# Autodesk Inventor assembly: 2016-02-05-RhinoRobotV10
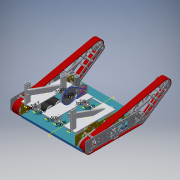
[picture p0: Inventor's stored thumbnail of the model, 180x180]
Saved by Autodesk Inventor 2016 SP1 (Build 200210100, 210)
## iProperties
Created: 2016-01-23
Part Number: 2016-02-05-RhinoRobotV10
Document SubType Name: Assembly
Designer: steele
Mass: 23360.3 g
Surface Area: 43274.3 cm^2
Volume: 23034.6 cm^3
Density: 1.01414 g/cm^3
Author: steele
## Documents named in this file (9)
- C:\snobotics\CAD-Development\robSteele\SnoBotics2016\2015-02-05-RhinoRobotNarrowView\2016-02-05-RhinoRobotV10.iam
- C:\snobotics\CAD-Development\robSteele\SnoBotics2016\RhinoTrackDriveModule\am-3322+RhinoTrackDriveModule.iam
- C:\snobotics\CAD-Development\robSteele\SnoBotics2016\RhinoBottomFloorOptions\RhinoBottomFloorPlate01.ipt
- C:\snobotics\CAD-Development\robSteele\SnoBotics2016\RhinoTrackDriveModule\am-3322+RhinoTrackDriveModule_MIR9.iam
- C:\snobotics\CAD-Development\robSteele\SnoBotics2016\AM Parts\Churo_16_5_inches.ipt
- C:\snobotics\CAD-Development\robSteele\SnoBotics2016\2016-01-31-Lift\ShortSupportPlateAssembly.iam
- C:\snobotics\CAD-Development\robSteele\SnoBotics2016\2015-02-05-RhinoRobotNarrowView\2016-02-05-RhinoRobotV10\Design Accelerator\Bolted Connection1.iam
- C:\snobotics\CAD-Development\robSteele\SnoBotics2016\2016-01-31-Lift\LongSupportPlateAssembly.iam
- C:\snobotics\CAD-Development\robSteele\SnoBotics2016\2016-01-31-Lift\ShortSupportPlateAssembly_MIR.iam
## Components (10 placed, 8 different names)
1. RhinoBottomFloorPlate01:1 — Mate:1, Flush:2, Flush:11
2. am-3322+RhinoTrackDriveModule:1 [sub-assembly] — Mate:1, Flush:2, Flush:11, Insert:1, Insert:2, Insert:6
3. am-3322+RhinoTrackDriveModule_MIR9:1 [sub-assembly]
4. Churo_16_5_inches:1 — Insert:1, Flush:18, Insert:7, Insert:9
5. Churo_16_5_inches:2 — Insert:2
6. Churo_16_5_inches:6 — Insert:6, Insert:8, Insert:10
7. ShortSupportPlateAssembly:1 [sub-assembly] — Insert:7, Insert:8, Mate:2, Mate:3
8. Bolted Connection:1 [sub-assembly] — Mate:2, Mate:3
9. LongSupportPlateAssembly:1 [sub-assembly] — Insert:9, Insert:10
10. ShortSupportPlateAssembly_MIR:1 [sub-assembly]
## Relationships (13: Insert 7, Mate 3, Flush 3)
- Mate:1: RhinoBottomFloorPlate01:1 ↔ am-3322+RhinoTrackDriveModule:1
- Flush:2: RhinoBottomFloorPlate01:1 ↔ am-3322+RhinoTrackDriveModule:1
- Flush:11: RhinoBottomFloorPlate01:1 ↔ am-3322+RhinoTrackDriveModule:1
- Insert:1: am-3322+RhinoTrackDriveModule:1 ↔ Churo_16_5_inches:1
- Insert:2: am-3322+RhinoTrackDriveModule:1 ↔ Churo_16_5_inches:2
- Insert:6: am-3322+RhinoTrackDriveModule:1 ↔ Churo_16_5_inches:6
- Flush:18: Churo_16_5_inches:1
- Insert:7: Churo_16_5_inches:1 ↔ ShortSupportPlateAssembly:1
- Insert:8: Churo_16_5_inches:6 ↔ ShortSupportPlateAssembly:1
- Insert:9 (-182.5625 mm): Churo_16_5_inches:1 ↔ LongSupportPlateAssembly:1
- Insert:10 (-182.5625 mm): Churo_16_5_inches:6 ↔ LongSupportPlateAssembly:1
- Mate:2: ShortSupportPlateAssembly:1 ↔ Bolted Connection:1
- Mate:3: ShortSupportPlateAssembly:1 ↔ Bolted Connection:1
## Named parameters: robotWidth = 660.4 mm, halfRobotWidth = 330.2 mm, maxPerimeter = 3048 mm, maxLength = 863.6 mm, widthOfTrack = 95.25 mm, boardWidth = 469.9 mm
